# Autodesk Inventor assembly: 尾翼
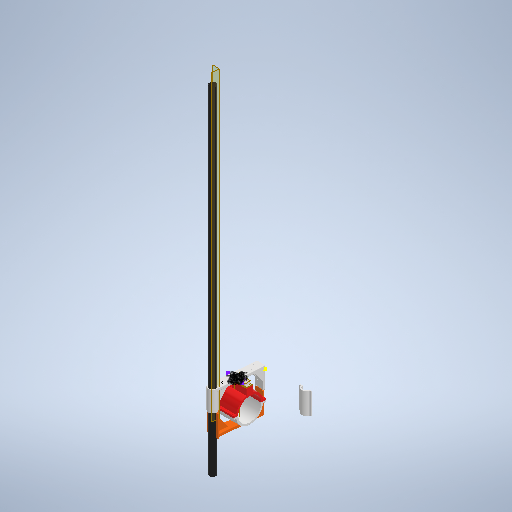
[picture p0: Inventor's stored thumbnail of the model, 512x512]
Saved by Autodesk Inventor 2025.2 (Build 292293000, 293)
## iProperties
Created: 2025-02-07
Part Number: 尾翼
Document SubType Name: Assembly
Designer: mahhy
Author: mahhy
## Documents named in this file (10)
- D:\兵庫県立大\部活\鳥人間部\尾翼.iam
- D:\兵庫県立大\部活\鳥人間部\motor-mount.ipt
- D:\兵庫県立大\部活\鳥人間部\moror-mount1.ipt
- D:\兵庫県立大\部活\鳥人間部\尾翼データ\servo_motor.ipt
- D:\兵庫県立大\部活\鳥人間部\arm-2.ipt
- D:\兵庫県立大\部活\鳥人間部\arm-2-2.ipt
- D:\兵庫県立大\部活\鳥人間部\尾翼データ\bearing.ipt
- D:\兵庫県立大\部活\鳥人間部\尾翼データ\pole.ipt
- C:\Users\mahhy\Downloads\ServoMotor_Hone2 (1).ipt
- D:\兵庫県立大\部活\鳥人間部\Part9.ipt
## Components (9 placed, 9 different names)
1. motor-mount:1 — リジッド:1, 挿入:6, メイト:5
2. moror-mount1:1 — リジッド:1, メイト:1, メイト:2, メイト:3
3. servo_motor:1 — 挿入:7, メイト:1, メイト:2, メイト:3
4. arm-2:1 — 挿入:8, 挿入:9
5. arm-2-2:1
6. bearing:1 — 挿入:6, 挿入:8
7. pole:1 — 挿入:9, 挿入:10
8. ServoMotor_Hone2 (1):1 — リジッド:3, 挿入:7
9. Part9:1 — リジッド:3, メイト:4, 挿入:10
## Relationships (12: Insert 5, Mate 5, WeldJoint 2)
- リジッド:1 [WeldJoint]: motor-mount:1 ↔ moror-mount1:1
- 挿入:6 [Insert]: motor-mount:1 ↔ bearing:1
- リジッド:3 [WeldJoint]: ServoMotor_Hone2 (1):1 ↔ Part9:1
- 挿入:7 [Insert]: servo_motor:1 ↔ ServoMotor_Hone2 (1):1
- メイト:1 [Mate]: moror-mount1:1 ↔ servo_motor:1
- メイト:2 [Mate]: moror-mount1:1 ↔ servo_motor:1
- メイト:3 [Mate]: moror-mount1:1 ↔ servo_motor:1
- 挿入:8 [Insert]: arm-2:1 ↔ bearing:1
- メイト:4 [Mate]: Part9:1
- メイト:5 [Mate]: motor-mount:1
- 挿入:9 [Insert] (-134 mm): arm-2:1 ↔ pole:1
- 挿入:10 [Insert] (1045.85 mm): pole:1 ↔ Part9:1
